# Autodesk Inventor assembly: Blade Assembly
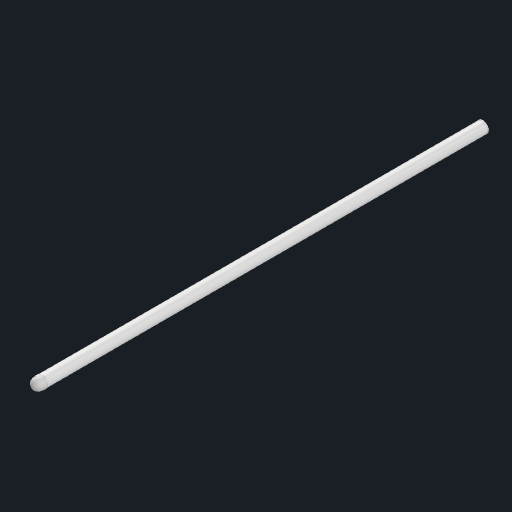
[picture p0: Inventor's stored thumbnail of the model, 512x512]
Saved by Autodesk Inventor 2022.2 (Build 262287000, 287)
## iProperties
Created: 2022-01-30
Part Number: Blade Assembly
Document SubType Name: Assembly
Designer: Michael Lacey
Mass: 438.646 g
Surface Area: 2773.17 cm^2
Volume: 392.14 cm^3
Density: 1.1186 g/cm^3
Author: Michael Lacey
## Documents named in this file (6)
- C:\Users\foams\3D Objects\Light Saber\assembly test components\Blade Assembly.iam
- C:\Users\foams\3D Objects\Light Saber\assembly test components\Shaft.ipt
- C:\Users\foams\3D Objects\Light Saber\assembly test components\EndCapblade.ipt
- C:\Users\foams\3D Objects\Light Saber\assembly test components\Diffusion Foam.ipt
- C:\Users\foams\3D Objects\Light Saber\assembly test components\PixelStick.ipt
- C:\Users\foams\3D Objects\Light Saber\assembly test components\Connector.ipt
## Components (5 placed, 5 different names)
1. Shaft:1 — Mate:1, Mate:2, Flush:1, Mate:3, Flush:2, Flush:3
2. EndCapblade:1 — Mate:1, Mate:2
3. Diffusion Foam:1 — Flush:1, Mate:3, Mate:4
4. PixelStick:1 — Mate:4, Flush:2
5. Connector:1 — Flush:3
## Relationships (7: Mate 4, Flush 3)
- Mate:1: Shaft:1 ↔ EndCapblade:1
- Mate:2: Shaft:1 ↔ EndCapblade:1
- Flush:1 (-38.1 mm): Shaft:1 ↔ Diffusion Foam:1
- Mate:3: Shaft:1 ↔ Diffusion Foam:1
- Mate:4: Diffusion Foam:1 ↔ PixelStick:1
- Flush:2 (25.4 mm): Shaft:1 ↔ PixelStick:1
- Flush:3: Shaft:1 ↔ Connector:1
